# Autodesk Inventor assembly: Tray
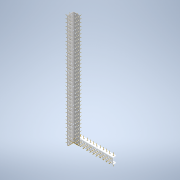
[picture p0: Inventor's stored thumbnail of the model, 180x180]
Saved by Autodesk Inventor 2020 (Build 240168000, 168)
## iProperties
Created: 2019-11-01
Part Number: Tray
Document SubType Name: Assembly
Designer: Alex Zaccardelli
Author: Alex Zaccardelli
## Documents named in this file (3)
- D:\DR4BTrayBot\Tray.iam
- D:\DR4BTrayBot\SIGBotsCADLibrary\Structure\C-Channel 2 x 12.ipt
- D:\DR4BTrayBot\SIGBotsCADLibrary\Structure\L-Channel 35 (aluminum).ipt
## Components (2 placed, 2 different names)
1. C-Channel 2 x 12:1 — Mate:1, Mate:2, Mate:3
2. L-Channel 35 (aluminum):1 — Mate:1, Mate:2, Mate:3
## Relationships (3: Mate 3)
- Mate:1: C-Channel 2 x 12:1 ↔ L-Channel 35 (aluminum):1
- Mate:2: C-Channel 2 x 12:1 ↔ L-Channel 35 (aluminum):1
- Mate:3: C-Channel 2 x 12:1 ↔ L-Channel 35 (aluminum):1
